# Autodesk Inventor assembly: hoop3_cog
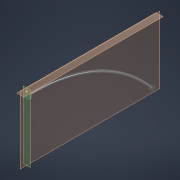
[picture p0: Inventor's stored thumbnail of the model, 180x180]
Saved by Autodesk Inventor 2021 (Build 250183000, 183)
## iProperties
Created: 2021-06-13
Part Number: hoop3_cog
Document SubType Name: Assembly
Designer: Watchdog
Mass: 1611.89 g
Surface Area: 2465.04 cm^2
Volume: 205.336 cm^3
Density: 7.85 g/cm^3
Author: Watchdog
## Documents named in this file (2)
- C:\Users\Watchdog\OneDrive - Flinders\Advn Mech Design Shared\6_Development\2_Design\inventor\hoop_slider\validationfiles\hoop3_cog.iam
- C:\Users\Watchdog\OneDrive - Flinders\Advn Mech Design Shared\6_Development\2_Design\inventor\hoop_slider\small_hoop.ipt
## Components (1 placed, 1 different names)
1. small_hoop:1 — Mate:1, Mate:2
## Relationships (2: Mate 2)
- Mate:1: small_hoop:1
- Mate:2: small_hoop:1
